# Autodesk Inventor assembly: CatchAssembly
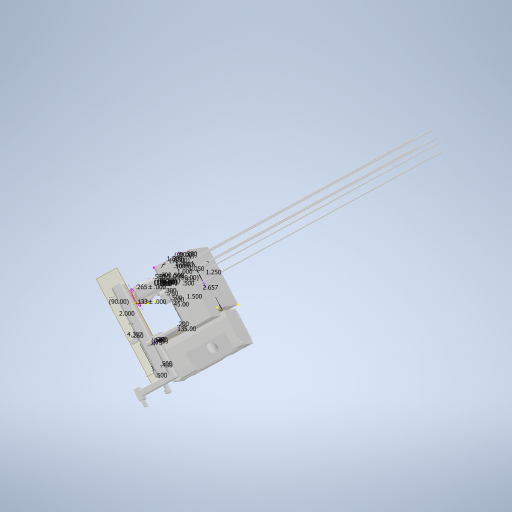
[picture p0: Inventor's stored thumbnail of the model, 512x512]
Saved by Autodesk Inventor 2024.1 (Build 281209000, 209)
## iProperties
Created: 2023-10-23
Part Number: CatchAssembly
Document SubType Name: Assembly
Designer: pab2
Author: pab2
## Documents named in this file (11)
- C:\Users\pab2\Documents\GitHub\AFL-hardware-devel\AFL-Platform\LoaderGen2\CatchAssembly.iam
- C:\Users\pab2\Documents\GitHub\AFL-hardware-devel\AFL-Platform\LoaderGen2\catch vertical seal-tighttol-thread - SANS.ipt
- C:\Users\pab2\Documents\GitHub\AFL-hardware-devel\AFL-Platform\LoaderGen2\CatchHolderNut.ipt
- C:\Users\pab2\Documents\GitHub\AFL-hardware-devel\AFL-Platform\LoaderGen2\Elevator arm r2.ipt
- C:\Users\pab2\Documents\GitHub\AFL-hardware-devel\AFL-Platform\LoaderGen2\full-up microswitch arm.ipt
- C:\Users\pab2\Documents\GitHub\AFL-hardware-devel\AFL-Platform\LoaderGen2\Valve Holder-3valve-withwirebox.ipt
- C:\Users\pab2\Documents\GitHub\AFL-hardware-devel\AFL-Platform\LoaderGen2\CatchlessCatchHolder-Braced-For1inCatch-Sidebar-Lowered.ipt
- C:\Users\pab2\Downloads\50185A34_Air-Powered Hold-Down Fixture Clamp\50185A34_Air-Powered Hold-Down Fixture Clamp.ipt
- C:\Users\pab2\Documents\GitHub\AFL-hardware-devel\AFL-Platform\LoaderGen2\piston badflowchannel-1-16in-thread - neutron - 65flowchan.ipt
- C:\Users\pab2\Downloads\5001T36_Miniature Solenoid On-Off Valve\5001T36_Miniature Solenoid On-Off Valve.ipt
- C:\Users\pab2\Downloads\8085T18_Subminiature Wet-Location Snap-Acting Switch\8085T18_Subminiature Wet-Location Snap-Acting Switch.ipt
## Components (13 placed, 10 different names)
1. catch vertical seal-tighttol-thread - SANS:1 — Mate:4, Mate:5, Mate:6, Mate:7, Mate:8, Mate:9, Insert:1
2. CatchHolderNut:1 — Mate:7, Mate:8, Mate:9
3. Elevator arm r2:1 — Mate:13, Mate:14
4. full-up microswitch arm:1 — Mate:15, Mate:16, Mate:17, Mate:18, Mate:19, Mate:20
5. Valve Holder-3valve-withwirebox:1 — Mate:10, Mate:11, Mate:12, Insert:2, Insert:3, Insert:4
6. CatchlessCatchHolder-Braced-For1inCatch-Sidebar-Lowered:1 — Mate:1, Mate:2, Mate:3, Mate:4, Mate:5, Mate:6, Mate:10, Mate:11, Mate:12, Mate:15, Mate:16, Mate:17, Mate:21, Mate:22, Mate:23
7. 50185A34_Air-Powered Hold-Down Fixture Clamp:1 — Mate:1, Mate:2, Mate:3, Mate:13, Mate:14
8. piston badflowchannel-1-16in-thread - neutron - 65flowchan:1 — Insert:1
9. 5001T36_Miniature Solenoid On-Off Valve:1 — Insert:3
10. 5001T36_Miniature Solenoid On-Off Valve:2 — Insert:2
11. 5001T36_Miniature Solenoid On-Off Valve:3 — Insert:4
12. 8085T18_Subminiature Wet-Location Snap-Acting Switch:1 — Mate:18, Mate:19, Mate:20
13. 8085T18_Subminiature Wet-Location Snap-Acting Switch:2 — Mate:21, Mate:22, Mate:23
## Relationships (27: Mate 23, Insert 4)
- Mate:1: CatchlessCatchHolder-Braced-For1inCatch-Sidebar-Lowered:1 ↔ 50185A34_Air-Powered Hold-Down Fixture Clamp:1
- Mate:2: CatchlessCatchHolder-Braced-For1inCatch-Sidebar-Lowered:1 ↔ 50185A34_Air-Powered Hold-Down Fixture Clamp:1
- Mate:3: CatchlessCatchHolder-Braced-For1inCatch-Sidebar-Lowered:1 ↔ 50185A34_Air-Powered Hold-Down Fixture Clamp:1
- Mate:4: catch vertical seal-tighttol-thread - SANS:1 ↔ CatchlessCatchHolder-Braced-For1inCatch-Sidebar-Lowered:1
- Mate:5: catch vertical seal-tighttol-thread - SANS:1 ↔ CatchlessCatchHolder-Braced-For1inCatch-Sidebar-Lowered:1
- Mate:6: catch vertical seal-tighttol-thread - SANS:1 ↔ CatchlessCatchHolder-Braced-For1inCatch-Sidebar-Lowered:1
- Mate:7: catch vertical seal-tighttol-thread - SANS:1 ↔ CatchHolderNut:1
- Mate:8: catch vertical seal-tighttol-thread - SANS:1 ↔ CatchHolderNut:1
- Mate:9: catch vertical seal-tighttol-thread - SANS:1 ↔ CatchHolderNut:1
- Mate:10: Valve Holder-3valve-withwirebox:1 ↔ CatchlessCatchHolder-Braced-For1inCatch-Sidebar-Lowered:1
- Mate:11: Valve Holder-3valve-withwirebox:1 ↔ CatchlessCatchHolder-Braced-For1inCatch-Sidebar-Lowered:1
- Mate:12: Valve Holder-3valve-withwirebox:1 ↔ CatchlessCatchHolder-Braced-For1inCatch-Sidebar-Lowered:1
- Mate:13: Elevator arm r2:1 ↔ 50185A34_Air-Powered Hold-Down Fixture Clamp:1
- Mate:14: Elevator arm r2:1 ↔ 50185A34_Air-Powered Hold-Down Fixture Clamp:1
- Mate:15: full-up microswitch arm:1 ↔ CatchlessCatchHolder-Braced-For1inCatch-Sidebar-Lowered:1
- Mate:16: full-up microswitch arm:1 ↔ CatchlessCatchHolder-Braced-For1inCatch-Sidebar-Lowered:1
- Mate:17: full-up microswitch arm:1 ↔ CatchlessCatchHolder-Braced-For1inCatch-Sidebar-Lowered:1
- Insert:1 (3.175 mm): catch vertical seal-tighttol-thread - SANS:1 ↔ piston badflowchannel-1-16in-thread - neutron - 65flowchan:1
- Insert:2: Valve Holder-3valve-withwirebox:1 ↔ 5001T36_Miniature Solenoid On-Off Valve:2
- Insert:3: Valve Holder-3valve-withwirebox:1 ↔ 5001T36_Miniature Solenoid On-Off Valve:1
- Insert:4: Valve Holder-3valve-withwirebox:1 ↔ 5001T36_Miniature Solenoid On-Off Valve:3
- Mate:18: full-up microswitch arm:1 ↔ 8085T18_Subminiature Wet-Location Snap-Acting Switch:1
- Mate:19: full-up microswitch arm:1 ↔ 8085T18_Subminiature Wet-Location Snap-Acting Switch:1
- Mate:20: full-up microswitch arm:1 ↔ 8085T18_Subminiature Wet-Location Snap-Acting Switch:1
- Mate:21: CatchlessCatchHolder-Braced-For1inCatch-Sidebar-Lowered:1 ↔ 8085T18_Subminiature Wet-Location Snap-Acting Switch:2
- Mate:22: CatchlessCatchHolder-Braced-For1inCatch-Sidebar-Lowered:1 ↔ 8085T18_Subminiature Wet-Location Snap-Acting Switch:2
- Mate:23: CatchlessCatchHolder-Braced-For1inCatch-Sidebar-Lowered:1 ↔ 8085T18_Subminiature Wet-Location Snap-Acting Switch:2
